# Autodesk Inventor assembly: 42T AM PULLY
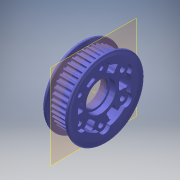
[picture p0: Inventor's stored thumbnail of the model, 180x180]
Saved by Autodesk Inventor 2019.4 (Build 234330000, 330)
## iProperties
Created: 2020-01-11
Part Number: 42T AM PULLY
Document SubType Name: Assembly
Designer: mavericks
Mass: 10.8862 g
Surface Area: 259.739 cm^2
Volume: 42.1139 cm^3
Density: 0.258494 g/cm^3
Author: mavericks
## Documents named in this file (2)
- T:\EIT\2020 Infinite Recharge\2020 ROBOT\COMMON PARTS\PULLEYS\htd\42T AM PULLY.iam
- T:\EIT\2020 Infinite Recharge\2020 ROBOT\COMMON PARTS\X - OTHER\am-2234_42toothHTDpulleyHalfRev2.ipt
## Components (2 placed, 1 different names)
1. am-2234_42toothHTDpulleyHalfRev2:1 — Insert:1, Insert:2, Symmetry:1
2. am-2234_42toothHTDpulleyHalfRev2:2 — Insert:1, Insert:2, Symmetry:1
## Relationships (3: Insert 2, Symmetry 1)
- Insert:1: am-2234_42toothHTDpulleyHalfRev2:1 ↔ am-2234_42toothHTDpulleyHalfRev2:2
- Insert:2: am-2234_42toothHTDpulleyHalfRev2:1 ↔ am-2234_42toothHTDpulleyHalfRev2:2
- Symmetry:1: am-2234_42toothHTDpulleyHalfRev2:1 ↔ am-2234_42toothHTDpulleyHalfRev2:2
